# Autodesk Inventor assembly: Assembly5
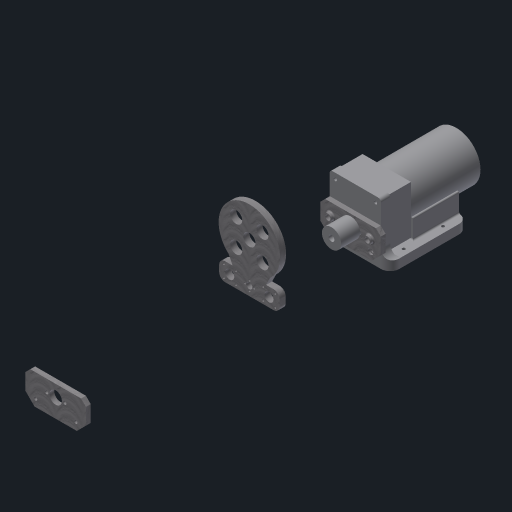
[picture p0: Inventor's stored thumbnail of the model, 512x512]
Saved by Autodesk Inventor 2024.3 (Build 283343000, 343)
## iProperties
Created: 2024-06-30
Part Number: Assembly5
Material: Generic
Document SubType Name: Assembly
Designer: Niler
Author: Niler
## Documents named in this file (6)
- C:\Users\Niler\OneDrive\Escritorio\RECICLADOR\RECICLADOR_MODELO_3D\CAJA_ENGRANAJES\VERSION_2\Assembly5.iam
- C:\Users\Niler\OneDrive\Escritorio\RECICLADOR\RECICLADOR_MODELO_3D\MECANISMO DE COMPACTADO\SOPORTE DEL MOTOR.ipt
- C:\Users\Niler\OneDrive\Escritorio\RECICLADOR\RECICLADOR_MODELO_3D\MECANISMO DE COMPACTADO\ACOPLE HELICOIDAL.ipt
- C:\Users\Niler\OneDrive\Escritorio\RECICLADOR\RECICLADOR_MODELO_3D\MECANISMO DE COMPACTADO\MOTOR DC.ipt
- C:\Users\Niler\OneDrive\Escritorio\RECICLADOR\RECICLADOR_MODELO_3D\CAJA_ENGRANAJES\VERSION_2\CAJA_V2.ipt
- C:\Users\Niler\OneDrive\Escritorio\RECICLADOR\RECICLADOR_MODELO_3D\CAJA_ENGRANAJES\VERSION_2\APLASTADOR.ipt
## Components (6 placed, 5 different names)
1. SOPORTE DEL MOTOR:1 — Mate:3, Angle:1, Mate:4, Mate:6, Mate:7
2. ACOPLE HELICOIDAL:1 — Mate:3, Mate:5, Mate:10
3. MOTOR DC:1 — Angle:1, Mate:4
4. CAJA_V2:1 — Mate:5, Mate:6, Mate:7, Mate:8, Mate:9, Mate:11
5. CAJA_V2:2 — Mate:8, Mate:9
6. APLASTADOR:1 — Mate:10, Mate:11
## Relationships (12: Mate 11, Angle 1)
- [Mate]: ACOPLE HELICOIDAL:1 ↔ MOTOR DC:1
- [Mate] (10 mm): ACOPLE HELICOIDAL:1 ↔ MOTOR DC:1
- Mate:3: SOPORTE DEL MOTOR:1 ↔ ACOPLE HELICOIDAL:1
- Angle:1 (0 deg): SOPORTE DEL MOTOR:1 ↔ MOTOR DC:1
- Mate:4: SOPORTE DEL MOTOR:1 ↔ MOTOR DC:1
- Mate:5: ACOPLE HELICOIDAL:1 ↔ CAJA_V2:1
- Mate:6: SOPORTE DEL MOTOR:1 ↔ CAJA_V2:1
- Mate:7: SOPORTE DEL MOTOR:1 ↔ CAJA_V2:1
- Mate:8: CAJA_V2:1 ↔ CAJA_V2:2
- Mate:9: CAJA_V2:1 ↔ CAJA_V2:2
- Mate:10: ACOPLE HELICOIDAL:1 ↔ APLASTADOR:1
- Mate:11: CAJA_V2:1 ↔ APLASTADOR:1
